# Autodesk Inventor assembly: Intake
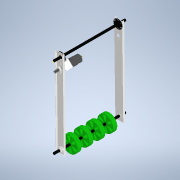
[picture p0: Inventor's stored thumbnail of the model, 180x180]
Saved by Autodesk Inventor 2021 (Build 250183000, 183)
## iProperties
Created: 2021-02-27
Part Number: Intake
Document SubType Name: Assembly
Designer: JavDiazV
Author: JavDiazV
## Documents named in this file (8)
- C:\Users\aidan\Desktop\T3 Robotics\CAD\2021 Specific Parts\Intake.iam
- C:\Users\aidan\Desktop\T3 Robotics\CAD\Javier's CAD\part_18 in. Thundershaft.ipt
- C:\Users\aidan\Desktop\T3 Robotics\CAD\Javier's CAD\part_4 in. Compliance Wheel.ipt
- C:\Users\aidan\Desktop\T3 Robotics\CAD\VerseFrame 18in C Channel.ipt
- C:\Users\aidan\Desktop\T3 Robotics\CAD\0.5in Hex Hub.ipt
- C:\Users\aidan\Desktop\T3 Robotics\CAD\Generic and Stock\VersaPlanetary Single Stage w 775.ipt
- C:\Users\aidan\Desktop\T3 Robotics\CAD\Bearing for THUNDER.ipt
- C:\Users\aidan\Desktop\T3 Robotics\CAD\Generic and Stock\16T 22 Sprocket.ipt
## Components (15 placed, 7 different names)
1. VerseFrame 18in C Channel:1 — Flush:1, Flush:2, Mate:1, Mate:3, Insert:16, Mate:10, Mate:14, Flush:10, Flush:11
2. VerseFrame 18in C Channel:2 — Flush:1, Flush:2, Mate:2, Mate:4, Mate:5, Mate:6, Mate:7, Mate:8, Insert:15, Mate:10, Mate:17
3. part_18 in. Thundershaft:1 — Mate:9, Angle:1, Flush:5, Mate:16, Angle:4, Mate:18, Mate:19
4. part_4 in. Compliance Wheel:1 — Mate:12, Flush:7, Flush:8
5. part_4 in. Compliance Wheel:2 — Mate:11, Mate:12, Flush:8, Flush:9
6. part_4 in. Compliance Wheel:3 — Mate:11, Mate:13, Flush:7, Mate:18, Mate:19
7. part_4 in. Compliance Wheel:4 — Mate:13, Flush:9, Flush:10
8. 0.5in Hex Hub:1 — Mate:2, Mate:4, Mate:5, Flush:3
9. 0.5in Hex Hub:2 — Mate:1, Mate:3, Flush:3, Angle:2
10. VersaPlanetary Single Stage w 775:1 — Mate:6, Mate:7, Mate:8, Mate:15, Angle:3
11. Bearing for THUNDER:1 — Insert:15, Flush:4, Mate:9
12. Bearing for THUNDER:2 — Insert:16, Flush:4, Angle:1, Flush:5
13. part_18 in. Thundershaft:2 — Mate:14, Angle:2, Flush:11
14. 16T 22 Sprocket:1 — Mate:15, Angle:3, Flush:6, Mate:17
15. 16T 22 Sprocket:2 — Mate:16, Angle:4, Flush:6
## Relationships (36: Mate 19, Flush 11, Angle 4, Insert 2)
- Flush:1: VerseFrame 18in C Channel:1 ↔ VerseFrame 18in C Channel:2
- Flush:2: VerseFrame 18in C Channel:1 ↔ VerseFrame 18in C Channel:2
- Mate:1: VerseFrame 18in C Channel:1 ↔ 0.5in Hex Hub:2
- Mate:2: VerseFrame 18in C Channel:2 ↔ 0.5in Hex Hub:1
- Mate:3: VerseFrame 18in C Channel:1 ↔ 0.5in Hex Hub:2
- Mate:4: VerseFrame 18in C Channel:2 ↔ 0.5in Hex Hub:1
- Mate:5: VerseFrame 18in C Channel:2 ↔ 0.5in Hex Hub:1
- Flush:3: 0.5in Hex Hub:1 ↔ 0.5in Hex Hub:2
- Mate:6: VerseFrame 18in C Channel:2 ↔ VersaPlanetary Single Stage w 775:1
- Mate:7: VerseFrame 18in C Channel:2 ↔ VersaPlanetary Single Stage w 775:1
- Mate:8: VerseFrame 18in C Channel:2 ↔ VersaPlanetary Single Stage w 775:1
- Insert:15: VerseFrame 18in C Channel:2 ↔ Bearing for THUNDER:1
- Insert:16: VerseFrame 18in C Channel:1 ↔ Bearing for THUNDER:2
- Flush:4: Bearing for THUNDER:1 ↔ Bearing for THUNDER:2
- Mate:9: part_18 in. Thundershaft:1 ↔ Bearing for THUNDER:1
- Angle:1 (0 deg): part_18 in. Thundershaft:1 ↔ Bearing for THUNDER:2
- Mate:10 (368.3 mm): VerseFrame 18in C Channel:1 ↔ VerseFrame 18in C Channel:2
- Flush:5 (31.75 mm): part_18 in. Thundershaft:1 ↔ Bearing for THUNDER:2
- Mate:11: part_4 in. Compliance Wheel:2 ↔ part_4 in. Compliance Wheel:3
- Mate:12: part_4 in. Compliance Wheel:1 ↔ part_4 in. Compliance Wheel:2
- Mate:13: part_4 in. Compliance Wheel:3 ↔ part_4 in. Compliance Wheel:4
- Mate:14: VerseFrame 18in C Channel:1 ↔ part_18 in. Thundershaft:2
- Angle:2 (0 deg): 0.5in Hex Hub:2 ↔ part_18 in. Thundershaft:2
- Mate:15: VersaPlanetary Single Stage w 775:1 ↔ 16T 22 Sprocket:1
- Angle:3 (0 deg): VersaPlanetary Single Stage w 775:1 ↔ 16T 22 Sprocket:1
- Mate:16: part_18 in. Thundershaft:1 ↔ 16T 22 Sprocket:2
- Angle:4 (0 deg): part_18 in. Thundershaft:1 ↔ 16T 22 Sprocket:2
- Flush:6: 16T 22 Sprocket:1 ↔ 16T 22 Sprocket:2
- Mate:17 (6.35 mm): VerseFrame 18in C Channel:2 ↔ 16T 22 Sprocket:1
- Flush:7 (76.2 mm): part_4 in. Compliance Wheel:1 ↔ part_4 in. Compliance Wheel:3
- Flush:8 (-76.2 mm): part_4 in. Compliance Wheel:1 ↔ part_4 in. Compliance Wheel:2
- Flush:9 (-76.2 mm): part_4 in. Compliance Wheel:2 ↔ part_4 in. Compliance Wheel:4
- Flush:10 (-88.9 mm): VerseFrame 18in C Channel:1 ↔ part_4 in. Compliance Wheel:4
- Mate:18: part_18 in. Thundershaft:1 ↔ part_4 in. Compliance Wheel:3
- Mate:19: part_18 in. Thundershaft:1 ↔ part_4 in. Compliance Wheel:3
- Flush:11 (43.18 mm): VerseFrame 18in C Channel:1 ↔ part_18 in. Thundershaft:2
